# Autodesk Inventor assembly: 武器把手
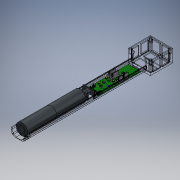
[picture p0: Inventor's stored thumbnail of the model, 180x180]
Saved by Autodesk Inventor 2017 (Build 210142000, 142)
## iProperties
Part Number: 武器把手
Material: 一般
Document SubType Name: Assembly
Designer: G
Author: G
## Documents named in this file (7)
- \\MissGAME-NAS\Miss GAME\松菸-幻影光靈\機關\武器把手\武器把手.iam
- \\MissGAME-NAS\Miss GAME\松菸-幻影光靈\機關\武器把手\手把A.ipt
- \\MissGAME-NAS\Miss GAME\松菸-幻影光靈\機關\武器把手\28650凸.ipt
- \\MissGAME-NAS\Miss GAME\松菸-幻影光靈\機關\武器把手\磁鐵A.ipt
- \\MissGAME-NAS\Miss GAME\松菸-幻影光靈\機關\武器把手\box.ipt
- \\MissGAME-NAS\Miss GAME\松菸-幻影光靈\機關\武器把手\電路板\電路板1.iam
- \\MissGAME-NAS\Miss GAME\松菸-幻影光靈\機關\武器把手\磁鐵b.ipt
## Components (7 placed, 6 different names)
1. box:2 — 貼合:5, 貼合:6, 貼合:8, 貼合:10, 貼合:11
2. 28650凸:1 — 貼合:2, 貼合:3, 貼合:8, 插入:1
3. 磁鐵A:1 — 貼合:4, 角度:2, 貼合:7, 貼合:11, 角度:3
4. 28650凸:2 — 插入:1
5. 手把A:2
6. 磁鐵b:1 — 貼合:2, 貼合:3, 貼合:4, 角度:2, 貼合:7
7. 電路板1:1 [sub-assembly] — 貼合:5, 貼合:6, 貼合:10, 角度:3
## Relationships (12: Mate 9, Angle 2, Insert 1)
- 貼合:2 [Mate]: 28650凸:1 ↔ 磁鐵b:1
- 貼合:3 [Mate] (5 mm): 28650凸:1 ↔ 磁鐵b:1
- 貼合:4 [Mate]: 磁鐵A:1 ↔ 磁鐵b:1
- 角度:2 [Angle] (0 deg): 磁鐵A:1 ↔ 磁鐵b:1
- 貼合:5 [Mate]: box:2 ↔ 電路板1:1
- 貼合:6 [Mate]: box:2 ↔ 電路板1:1
- 貼合:7 [Mate]: 磁鐵A:1 ↔ 磁鐵b:1
- 貼合:8 [Mate]: box:2 ↔ 28650凸:1
- 貼合:10 [Mate]: box:2 ↔ 電路板1:1
- 插入:1 [Insert]: 28650凸:1 ↔ 28650凸:2
- 貼合:11 [Mate] (0.1 mm): box:2 ↔ 磁鐵A:1
- 角度:3 [Angle] (0 deg): 磁鐵A:1 ↔ 電路板1:1
